# Autodesk Inventor assembly: X9X
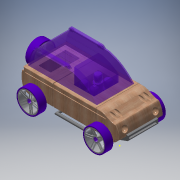
[picture p0: Inventor's stored thumbnail of the model, 180x180]
Saved by Autodesk Inventor 2018 (Build 220112000, 112)
## iProperties
Created: 2018-02-20
Part Number: X9X
Document SubType Name: Assembly
Designer: Blue Mist
Author: Blue Mist
## Documents named in this file (8)
- C:\Users\Tudor Mironovici\Documents\School\12th grade\Intro to Engineering\Automoblox X9X Project\X9X.iam
- C:\Users\Tudor Mironovici\Documents\School\12th grade\Intro to Engineering\Automoblox X9X Project\X9X Back.ipt
- C:\Users\Tudor Mironovici\Documents\School\12th grade\Intro to Engineering\Automoblox X9X Project\X9X Middle.ipt
- C:\Users\Tudor Mironovici\Documents\School\12th grade\Intro to Engineering\Automoblox X9X Project\X9X Front.ipt
- C:\Users\Tudor Mironovici\Documents\School\12th grade\Intro to Engineering\Automoblox X9X Project\X9X Windshield.ipt
- C:\Users\Tudor Mironovici\Documents\School\12th grade\Intro to Engineering\Automoblox X9X Project\X9X Rim.ipt
- C:\Users\Tudor Mironovici\Documents\School\12th grade\Intro to Engineering\Automoblox X9X Project\X9X Tire.ipt
- C:\Users\Tudor Mironovici\Documents\School\12th grade\Intro to Engineering\Automoblox X9X Project\X9X Person.ipt
## Components (18 placed, 7 different names)
1. X9X Back:1 — Rigid:1, Rotational:11, Rotational:14, Rotational:15
2. X9X Middle:1 — Rigid:1, Rigid:2, Rigid:3, Mate:1, Mate:2, Mate:3, Mate:4
3. X9X Front:1 — Rigid:2, Rotational:12, Rotational:13
4. X9X Windshield:1 — Rigid:3
5. X9X Rim:6 — Rotational:11, Rotational:17
6. X9X Rim:7 — Rotational:12, Rotational:18
7. X9X Rim:8 — Rotational:15, Rotational:21
8. X9X Rim:9 — Rotational:13, Rotational:20
9. X9X Rim:10 — Rotational:14, Rotational:19
10. X9X Tire:2 — Rotational:17
11. X9X Tire:3 — Rotational:18
12. X9X Tire:4 — Rotational:19
13. X9X Tire:5 — Rotational:20
14. X9X Tire:6 — Rotational:21
15. X9X Person:1 — Mate:4
16. X9X Person:2 — Mate:3
17. X9X Person:3 — Mate:2
18. X9X Person:4 — Mate:1
## Relationships (17: RevoluteJoint 10, Mate 4, WeldJoint 3)
- Rigid:1 [WeldJoint]: X9X Back:1 ↔ X9X Middle:1
- Rigid:2 [WeldJoint]: X9X Middle:1 ↔ X9X Front:1
- Rigid:3 [WeldJoint]: X9X Middle:1 ↔ X9X Windshield:1
- Rotational:11 [RevoluteJoint]: X9X Back:1 ↔ X9X Rim:6
- Rotational:12 [RevoluteJoint]: X9X Front:1 ↔ X9X Rim:7
- Rotational:13 [RevoluteJoint]: X9X Front:1 ↔ X9X Rim:9
- Rotational:14 [RevoluteJoint]: X9X Back:1 ↔ X9X Rim:10
- Rotational:15 [RevoluteJoint]: X9X Back:1 ↔ X9X Rim:8
- Rotational:17 [RevoluteJoint]: X9X Rim:6 ↔ X9X Tire:2
- Rotational:18 [RevoluteJoint]: X9X Rim:7 ↔ X9X Tire:3
- Rotational:19 [RevoluteJoint]: X9X Rim:10 ↔ X9X Tire:4
- Rotational:20 [RevoluteJoint]: X9X Rim:9 ↔ X9X Tire:5
- Rotational:21 [RevoluteJoint]: X9X Rim:8 ↔ X9X Tire:6
- Mate:1: X9X Middle:1 ↔ X9X Person:4
- Mate:2: X9X Middle:1 ↔ X9X Person:3
- Mate:3: X9X Middle:1 ↔ X9X Person:2
- Mate:4: X9X Middle:1 ↔ X9X Person:1
